# Autodesk Inventor assembly: chamber_with_holder
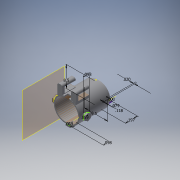
[picture p0: Inventor's stored thumbnail of the model, 180x180]
Saved by Autodesk Inventor 2016 (Build 200138000, 138)
## iProperties
Created: 2016-08-11
Part Number: chamber_with_holder
Document SubType Name: Weldment
Designer: GentnerLab
Weld Material: Welded Aluminum-6061
Author: GentnerLab
## Documents named in this file (7)
- C:\Users\GentnerLab\Documents\Inventor\Parts\new_drive\60unm-6mm\chamber_with_holder.iam
- C:\Users\GentnerLab\Documents\Inventor\Parts\new_drive\60unm-6mm\chamber_10mm.ipt
- C:\Users\GentnerLab\Documents\Inventor\Parts\new_drive\60unm-6mm\chamber_conn_holder.ipt
- C:\Users\GentnerLab\Documents\Inventor\Parts\new_drive\60unm-6mm\chamber_conn_holder_MIR.ipt
- C:\Users\GentnerLab\Documents\Inventor\Parts\new_drive\60unm-6mm\nail.ipt
- C:\Users\GentnerLab\Documents\Inventor\Parts\new_drive\60unm-6mm\nail_MIR1.ipt
- C:\Users\GentnerLab\Documents\GentnerLabSTL\Part2.ipt
## Components (7 placed, 6 different names)
1. chamber_10mm:1 — Mate:1, Mate:4, Mate:5, Mate:6, Tangent:1, Mate:17, Flush:4
2. chamber_conn_holder:1 — Mate:2, Mate:4
3. chamber_conn_holder_MIR:1 — Mate:7
4. nail:1 — Mate:15
5. nail_MIR1:1 — Mate:16
6. nail:2 — Mate:20
7. Part2:1 — Flush:4
## Relationships (22: Mate 16, Angle 3, Flush 2, Tangent 1)
- Mate:1: chamber_10mm:1
- Mate:2: chamber_conn_holder:1
- Mate:4 (2.75 mm): chamber_10mm:1 ↔ chamber_conn_holder:1
- Mate:5: chamber_10mm:1
- Angle:1 (0 deg)
- Mate:6: chamber_10mm:1
- Angle:2 (0 deg)
- Mate:7: chamber_conn_holder_MIR:1
- Angle:3 (0 deg)
- Tangent:1: chamber_10mm:1
- Mate:8
- Mate:9
- Flush:3 (2 mm)
- Mate:13
- Mate:14
- Mate:15: nail:1
- Mate:16: nail_MIR1:1
- Mate:17: chamber_10mm:1
- Mate:18
- Mate:19
- Mate:20 (0.25 mm): nail:2
- Flush:4: chamber_10mm:1 ↔ Part2:1
